# Autodesk Inventor assembly: assy_curved_right
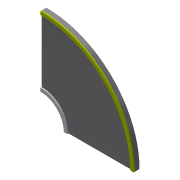
[picture p0: Inventor's stored thumbnail of the model, 180x180]
Saved by Autodesk Inventor 2018 (Build 220112000, 112)
## iProperties
Created: 2017-11-13
Part Number: assy_curved_right
Document SubType Name: Assembly
Designer: Platform
Author: Platform
## Documents named in this file (4)
- C:\Users\Platform\Desktop\autorace_track\track_model\autorace_rbizchallenge2017\assembled\assy_curved_right.iam
- C:\Users\Platform\Desktop\autorace_track\track_model\autorace_rbizchallenge2017\parts\ipt\upper_plate_curve v1.ipt
- C:\Users\Platform\Desktop\autorace_track\track_model\autorace_rbizchallenge2017\parts\ipt\curved_line_big.ipt
- C:\Users\Platform\Desktop\autorace_track\track_model\autorace_rbizchallenge2017\parts\ipt\curved_line_sml.ipt
## Components (3 placed, 3 different names)
1. upper_plate_curve v1:1
2. curved_line_big:1
3. curved_line_sml:1
## Relationships (3: Mate 3)
- [Mate]: upper_plate_curve v1:1 ↔ curved_line_big:1
- [Mate]: upper_plate_curve v1:1 ↔ curved_line_big:1
- [Mate]: upper_plate_curve v1:1 ↔ curved_line_sml:1
